# Autodesk Inventor assembly: Collector Arms v2.0_MIR_MIR
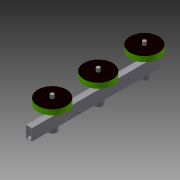
[picture p0: Inventor's stored thumbnail of the model, 180x180]
Saved by Autodesk Inventor 2015 (Build 190159000, 159)
## iProperties
Created: 2015-01-20
Part Number: Collector Arms v2.0_MIR_MIR
Document SubType Name: Assembly
Designer: chapale16
Author: chapale16
## Documents named in this file (4)
- \\lhssvr02\Homedirs\Robotics Club\CAD Model 2015\Game Components\The Tote Collector-Arms\Collector Arms v2.0_MIR_MIR.iam
- \\lhssvr02\Homedirs\Robotics Club\CAD Model 2015\Game Components\The Tote Collector-Arms\23.5 in 2 x 1 boxBeam_MIR_MIR.ipt
- \\lhssvr02\Homedirs\Robotics Club\CAD Model 2015\Game Components\The Tote Collector-Arms\P60 Gear Box_MIR2_MIR.ipt
- \\lhssvr02\Homedirs\Robotics Club\CAD Model 2015\Game Components\The Tote Collector-Arms\collector arm wheel_MIR2_MIR.ipt
## Components (7 placed, 3 different names)
1. 23.5 in 2 x 1 boxBeam_MIR_MIR:1 — Flush:1, Mate:1, Mate:5, Flush:3, Mate:8, Flush:5, Flush:9
2. P60 Gear Box_MIR2_MIR:1 — Flush:1, Mate:1, Mate:2, Flush:9, Mate:11
3. collector arm wheel_MIR2_MIR:1 — Mate:2, Flush:4
4. P60 Gear Box_MIR2_MIR:2 — Mate:5, Flush:3, Mate:3, Mate:10, Mate:11
5. collector arm wheel_MIR2_MIR:2 — Mate:3, Flush:4, Flush:6
6. P60 Gear Box_MIR2_MIR:3 — Mate:8, Flush:5, Mate:6, Mate:10
7. collector arm wheel_MIR2_MIR:3 — Mate:6, Flush:6
## Relationships (14: Mate 8, Flush 6)
- Flush:1: 23.5 in 2 x 1 boxBeam_MIR_MIR:1 ↔ P60 Gear Box_MIR2_MIR:1
- Mate:1: 23.5 in 2 x 1 boxBeam_MIR_MIR:1 ↔ P60 Gear Box_MIR2_MIR:1
- Mate:2: P60 Gear Box_MIR2_MIR:1 ↔ collector arm wheel_MIR2_MIR:1
- Mate:5: 23.5 in 2 x 1 boxBeam_MIR_MIR:1 ↔ P60 Gear Box_MIR2_MIR:2
- Flush:3: 23.5 in 2 x 1 boxBeam_MIR_MIR:1 ↔ P60 Gear Box_MIR2_MIR:2
- Mate:3: P60 Gear Box_MIR2_MIR:2 ↔ collector arm wheel_MIR2_MIR:2
- Flush:4: collector arm wheel_MIR2_MIR:1 ↔ collector arm wheel_MIR2_MIR:2
- Mate:8: 23.5 in 2 x 1 boxBeam_MIR_MIR:1 ↔ P60 Gear Box_MIR2_MIR:3
- Flush:5: 23.5 in 2 x 1 boxBeam_MIR_MIR:1 ↔ P60 Gear Box_MIR2_MIR:3
- Mate:6: P60 Gear Box_MIR2_MIR:3 ↔ collector arm wheel_MIR2_MIR:3
- Flush:6: collector arm wheel_MIR2_MIR:2 ↔ collector arm wheel_MIR2_MIR:3
- Flush:9 (114.3 mm): 23.5 in 2 x 1 boxBeam_MIR_MIR:1 ↔ P60 Gear Box_MIR2_MIR:1
- Mate:10 (161.3154 mm): P60 Gear Box_MIR2_MIR:2 ↔ P60 Gear Box_MIR2_MIR:3
- Mate:11 (161.3154 mm): P60 Gear Box_MIR2_MIR:1 ↔ P60 Gear Box_MIR2_MIR:2
